# Autodesk Inventor assembly: 9417K611_Gas Spring
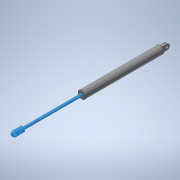
[picture p0: Inventor's stored thumbnail of the model, 180x180]
Saved by Autodesk Inventor 2020 (Build 240168000, 168)
## iProperties
Created: 2022-01-30
Part Number: 9417K611_Gas Spring
Document SubType Name: Assembly
Designer: mavericks
Author: mavericks
## Documents named in this file (3)
- T:\EIT\2022 Rapid React\COMMON PARTS\MCMASTER\Gas spring\9417K611_Gas Spring.iam
- T:\EIT\2022 Rapid React\COMMON PARTS\MCMASTER\Solid1.ipt
- T:\EIT\2022 Rapid React\COMMON PARTS\MCMASTER\Solid2.ipt
## Components (2 placed, 2 different names)
1. Solid1:1 — Mate:1, Angle:1, Mate:2
2. Solid2:1 — Mate:1, Angle:1, Mate:2
## Relationships (3: Mate 2, Angle 1)
- Mate:1: Solid1:1 ↔ Solid2:1
- Angle:1 (0 deg): Solid1:1 ↔ Solid2:1
- Mate:2: Solid1:1 ↔ Solid2:1
